# Autodesk Inventor assembly: PMT Re-entrant Flange
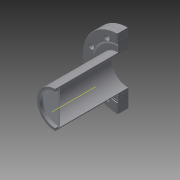
[picture p0: Inventor's stored thumbnail of the model, 180x180]
Saved by Autodesk Inventor 2015 (Build 190159000, 159)
## iProperties
Created: 2014-07-10
Part Number: PMT Re-entrant Flange
Document SubType Name: Assembly
Designer: I Rabey
Author: I Rabey
## Documents named in this file (5)
- C:\ColdMatter\CADFiles\EDM Machine\Microwave Detection Region\Re-entrant Flange\PMT Re-entrant Flange.iam
- C:\ColdMatter\CADFiles\EDM Machine\Microwave Detection Region\Re-entrant Flange\DN63CF Counter Bored.ipt
- C:\ColdMatter\CADFiles\EDM Machine\Microwave Detection Region\Re-entrant Flange\Vacuum Cylinder.ipt
- C:\ColdMatter\CADFiles\EDM Machine\Microwave Detection Region\Re-entrant Flange\PMT Cap.ipt
- C:\ColdMatter\CADFiles\EDM Machine\Microwave Detection Region\Re-entrant Flange\Window.ipt
## Components (4 placed, 4 different names)
1. DN63CF Counter Bored:1 — Mate:1, Mate:2, Mate:3, Mate:4
2. Vacuum Cylinder:1 — Mate:3, Mate:4, Mate:5, Mate:6, Mate:7
3. PMT Cap:1 — Mate:5, Mate:6, Mate:8, Angle:1
4. Window:1 — Mate:7, Mate:8
## Relationships (9: Mate 8, Angle 1)
- Mate:1: DN63CF Counter Bored:1
- Mate:2: DN63CF Counter Bored:1
- Mate:3: DN63CF Counter Bored:1 ↔ Vacuum Cylinder:1
- Mate:4: DN63CF Counter Bored:1 ↔ Vacuum Cylinder:1
- Mate:5: Vacuum Cylinder:1 ↔ PMT Cap:1
- Mate:6: Vacuum Cylinder:1 ↔ PMT Cap:1
- Mate:7: Vacuum Cylinder:1 ↔ Window:1
- Mate:8: PMT Cap:1 ↔ Window:1
- Angle:1 (45 deg): PMT Cap:1
